# Autodesk Inventor assembly: 240626_chairA
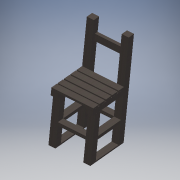
[picture p0: Inventor's stored thumbnail of the model, 180x180]
Saved by Autodesk Inventor 2016 (Build 200138000, 138)
## iProperties
Created: 2024-06-26
Part Number: 240626_chairA
Material: 일반
Document SubType Name: Assembly
Designer: pc
Author: pc
## Documents named in this file (8)
- D:\CAD_HCH\240626\240626_chairA.iam
- D:\CAD_HCH\240626\240626_chair1.ipt
- D:\CAD_HCH\240626\240626_chair2.ipt
- D:\CAD_HCH\240626\240626_chair3.ipt
- D:\CAD_HCH\240626\240626_chair4.ipt
- D:\CAD_HCH\240626\240626_chair5.ipt
- D:\CAD_HCH\240626\240626_chair6.ipt
- D:\CAD_HCH\240626\240626_chair7.ipt
## Components (18 placed, 7 different names)
1. 240626_chair2:1 — 메이트:1, 플러쉬:1, 플러쉬:2, 메이트:3, 플러쉬:7, 플러쉬:8, 메이트:14
2. 240626_chair2:2 — 메이트:2, 플러쉬:3, 플러쉬:4, 플러쉬:5, 플러쉬:6, 메이트:5
3. 240626_chair3:1 — 플러쉬:5, 플러쉬:6, 플러쉬:10, 메이트:5, 메이트:7, 플러쉬:11, 메이트:10, 플러쉬:15, 플러쉬:16, 플러쉬:18, 플러쉬:19
4. 240626_chair3:2 — 메이트:3, 플러쉬:7, 플러쉬:8, 메이트:6, 메이트:8, 플러쉬:12, 메이트:9, 플러쉬:13, 플러쉬:14
5. 240626_chair4:1 — 플러쉬:10, 메이트:6
6. 240626_chair4:2 — 메이트:8, 플러쉬:12, 플러쉬:22
7. 240626_chair4:3 — 메이트:7, 플러쉬:11
8. 240626_chair5:1 — 메이트:9, 플러쉬:13, 플러쉬:14, 메이트:13, 메이트:15
9. 240626_chair5:2 — 메이트:10, 플러쉬:15, 플러쉬:16, 메이트:11, 플러쉬:17, 플러쉬:18, 플러쉬:19
10. 240626_chair6:1 — 메이트:11, 메이트:12, 플러쉬:17, 메이트:16, 메이트:17
11. 240626_chair6:2 — 메이트:13, 메이트:14, 메이트:15, 플러쉬:20, 플러쉬:21, 플러쉬:22
12. 240626_chair7:1 — 메이트:16, 플러쉬:20
13. 240626_chair4:4 — 메이트:17, 플러쉬:21
14. 240626_chair1:1 — 메이트:1, 플러쉬:1, 플러쉬:2, 메이트:2, 플러쉬:3, 플러쉬:4
15. 240626_chair1:2
16. 240626_chair1:3
17. 240626_chair1:4
18. 240626_chair1:5 — 메이트:12
## Component patterns: (5 elements, first: 240626_chair1:1)
## Relationships (37: Flush 21, Mate 16)
- 메이트:1 [Mate]: 240626_chair2:1 ↔ 240626_chair1:1
- 플러쉬:1 [Flush]: 240626_chair2:1 ↔ 240626_chair1:1
- 플러쉬:2 [Flush]: 240626_chair2:1 ↔ 240626_chair1:1
- 메이트:2 [Mate]: 240626_chair2:2 ↔ 240626_chair1:1
- 플러쉬:3 [Flush]: 240626_chair2:2 ↔ 240626_chair1:1
- 플러쉬:4 [Flush]: 240626_chair2:2 ↔ 240626_chair1:1
- 플러쉬:5 [Flush]: 240626_chair2:2 ↔ 240626_chair3:1
- 플러쉬:6 [Flush] (5 mm): 240626_chair2:2 ↔ 240626_chair3:1
- 메이트:3 [Mate]: 240626_chair2:1 ↔ 240626_chair3:2
- 플러쉬:7 [Flush]: 240626_chair2:1 ↔ 240626_chair3:2
- 플러쉬:8 [Flush] (5 mm): 240626_chair2:1 ↔ 240626_chair3:2
- 플러쉬:10 [Flush] (-30 mm): 240626_chair3:1 ↔ 240626_chair4:1
- 메이트:5 [Mate]: 240626_chair2:2 ↔ 240626_chair3:1
- 메이트:6 [Mate]: 240626_chair3:2 ↔ 240626_chair4:1
- 메이트:7 [Mate]: 240626_chair3:1 ↔ 240626_chair4:3
- 플러쉬:11 [Flush] (30 mm): 240626_chair3:1 ↔ 240626_chair4:3
- 메이트:8 [Mate]: 240626_chair3:2 ↔ 240626_chair4:2
- 플러쉬:12 [Flush] (30 mm): 240626_chair3:2 ↔ 240626_chair4:2
- 메이트:9 [Mate]: 240626_chair3:2 ↔ 240626_chair5:1
- 플러쉬:13 [Flush]: 240626_chair3:2 ↔ 240626_chair5:1
- 플러쉬:14 [Flush]: 240626_chair3:2 ↔ 240626_chair5:1
- 메이트:10 [Mate]: 240626_chair3:1 ↔ 240626_chair5:2
- 플러쉬:15 [Flush]: 240626_chair3:1 ↔ 240626_chair5:2
- 플러쉬:16 [Flush]: 240626_chair3:1 ↔ 240626_chair5:2
- 메이트:11 [Mate]: 240626_chair5:2 ↔ 240626_chair6:1
- 메이트:12 [Mate]: 240626_chair6:1 ↔ 240626_chair1:5
- 플러쉬:17 [Flush]: 240626_chair5:2 ↔ 240626_chair6:1
- 플러쉬:18 [Flush]: 240626_chair3:1 ↔ 240626_chair5:2
- 플러쉬:19 [Flush]: 240626_chair3:1 ↔ 240626_chair5:2
- 메이트:13 [Mate]: 240626_chair5:1 ↔ 240626_chair6:2
- 메이트:14 [Mate]: 240626_chair2:1 ↔ 240626_chair6:2
- 메이트:15 [Mate]: 240626_chair5:1 ↔ 240626_chair6:2
- 메이트:16 [Mate]: 240626_chair6:1 ↔ 240626_chair7:1
- 플러쉬:20 [Flush] (20 mm): 240626_chair6:2 ↔ 240626_chair7:1
- 메이트:17 [Mate]: 240626_chair6:1 ↔ 240626_chair4:4
- 플러쉬:21 [Flush]: 240626_chair6:2 ↔ 240626_chair4:4
- 플러쉬:22 [Flush]: 240626_chair4:2 ↔ 240626_chair6:2
